# Autodesk Inventor assembly: Assembly_panel
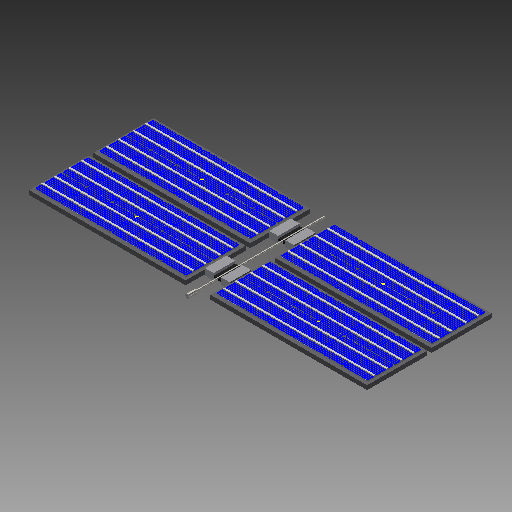
[picture p0: Inventor's stored thumbnail of the model, 512x512]
Saved by Autodesk Inventor 2018 (Build 220112000, 112)
## iProperties
Created: 2021-03-17
Part Number: Assembly_panel
Document SubType Name: Assembly
Designer: Patel
Author: Patel
## Documents named in this file (4)
- C:\Users\dell\Desktop\ES101 PROJECT\INDIVIDUAL MODELS\Kush\Assembly_panel.iam
- C:\Users\dell\Desktop\ES101 PROJECT\INDIVIDUAL MODELS\Kush\Rod.ipt
- C:\Users\dell\Desktop\ES101 PROJECT\INDIVIDUAL MODELS\Kush\Solar_panel1.ipt
- C:\Users\dell\Desktop\ES101 PROJECT\INDIVIDUAL MODELS\Kush\Solar_panel1_MIR.ipt
## Components (5 placed, 3 different names)
1. Rod:1 — Rigid:1, Rigid:2, Flush:1
2. Solar_panel1:1 — Rigid:1
3. Solar_panel1:3 — Rigid:2
4. Solar_panel1_MIR:1
5. Solar_panel1_MIR:2
## Relationships (3: WeldJoint 2, Flush 1)
- Rigid:1 [WeldJoint]: Rod:1 ↔ Solar_panel1:1
- Rigid:2 [WeldJoint]: Rod:1 ↔ Solar_panel1:3
- Flush:1 (-150 mm): Rod:1
